# Autodesk Inventor assembly: beczka1
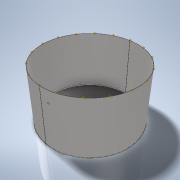
[picture p0: Inventor's stored thumbnail of the model, 180x180]
Saved by Autodesk Inventor 2021 (Build 250183000, 183)
## iProperties
Created: 2021-09-19
Part Number: beczka1
Document SubType Name: Weldment
Designer: wojwo
Weld Material: Welded Aluminum-6061
Author: wojwo
## Documents named in this file (4)
- D:\OneDrive\Documents\autodesk\beczka\beczka1.iam
- D:\OneDrive\Documents\autodesk\beczka\floor1.ipt
- D:\OneDrive\Documents\autodesk\beczka\fllooor22.ipt
- D:\OneDrive\Documents\autodesk\beczka\bok2137.ipt
## Components (3 placed, 3 different names)
1. floor1:1 — Zestawiające:1, Zestawiające:2, Zestawiające:3
2. fllooor22:1 — Zestawiające:4, Równoległe:1, Zestawiające:5
3. bok2137:1 — Równoległe:2
## Relationships (7: Mate 5, Flush 2)
- Zestawiające:1 [Mate]: floor1:1
- Zestawiające:2 [Mate]: floor1:1
- Zestawiające:3 [Mate]: floor1:1
- Zestawiające:4 [Mate]: fllooor22:1
- Równoległe:1 [Flush]: fllooor22:1
- Zestawiające:5 [Mate]: fllooor22:1
- Równoległe:2 [Flush]: bok2137:1
